# Autodesk Inventor assembly: LaundryRobot_v01
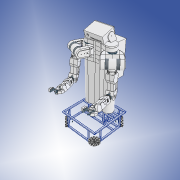
[picture p0: Inventor's stored thumbnail of the model, 180x180]
Saved by Autodesk Inventor 2017 (Build 210142000, 142)
## iProperties
Created: 2017-03-11
Part Number: LaundryRobot_v01
Document SubType Name: Assembly
Designer: zallen
Author: zallen
## Documents named in this file (4)
- C:\Users\zallen\Documents\GitHub\cr-laundry-robot\LaundryRobot_v01.iam
- C:\Users\zallen\Documents\GitHub\cr-laundry-robot\src\Body\Body.iam
- C:\Users\zallen\Documents\GitHub\cr-laundry-robot\src\Head\Head.iam
- C:\Users\zallen\Documents\GitHub\cr-laundry-robot\src\Base 2\Base2.iam
## Components (3 placed, 3 different names)
1. Body:1 [sub-assembly] — Mate:7, Mate:18, Mate:20
2. Head:1 [sub-assembly] — Mate:7, Mate:18, Mate:20
3. Base2:1 [sub-assembly] — Mate:11, Mate:12
## Relationships (5: Mate 5)
- Mate:7: Body:1 ↔ Head:1
- Mate:11: Base2:1
- Mate:12: Base2:1
- Mate:18: Body:1 ↔ Head:1
- Mate:20: Body:1 ↔ Head:1
